# Autodesk Inventor assembly: FulBotV2P1
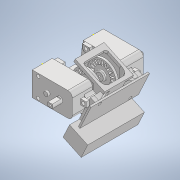
[picture p0: Inventor's stored thumbnail of the model, 180x180]
Saved by Autodesk Inventor 2022 (Build 260153070, 153G)
## iProperties
Created: 2022-02-15
Part Number: FulBotV2P1
Document SubType Name: Assembly
Designer: a laptop
Author: a laptop
## Documents named in this file (6)
- C:\Users\a laptop\Desktop\SumoBot\FulBotV2P1.iam
- C:\Users\a laptop\Desktop\SumoBot\sumobotENCODER\EncoderV2\EncoderV2.5.iam
- C:\Users\a laptop\Desktop\SumoBot\REF_PART\2sLIPO_SMALLER.ipt
- C:\Users\a laptop\Desktop\SumoBot\sumobotENCODER\EncoderV2\EncoderV2.5_MIR.iam
- C:\Users\a laptop\Desktop\SumoBot\REF_PART\XL4015.ipt
- C:\Users\a laptop\Desktop\SumoBot\sumobotFRAME\Encoderconnector.ipt
## Components (5 placed, 5 different names)
1. EncoderV2.5:1 [sub-assembly] — Flush:2, Flush:3, Mate:1, Mate:4
2. 2sLIPO_SMALLER:1 — Mate:3
3. EncoderV2.5_MIR:1 [sub-assembly] — Flush:2, Flush:3, Mate:2
4. XL4015:1 — Mate:5, Mate:6, Mate:7
5. Encoderconnector:1 — Mate:1, Mate:2, Mate:3, Mate:4, Mate:5, Mate:6, Mate:7
## Relationships (9: Mate 7, Flush 2)
- Flush:2: EncoderV2.5:1 ↔ EncoderV2.5_MIR:1
- Flush:3: EncoderV2.5:1 ↔ EncoderV2.5_MIR:1
- Mate:1: EncoderV2.5:1 ↔ Encoderconnector:1
- Mate:2: EncoderV2.5_MIR:1 ↔ Encoderconnector:1
- Mate:3: 2sLIPO_SMALLER:1 ↔ Encoderconnector:1
- Mate:4: EncoderV2.5:1 ↔ Encoderconnector:1
- Mate:5: XL4015:1 ↔ Encoderconnector:1
- Mate:6: XL4015:1 ↔ Encoderconnector:1
- Mate:7: XL4015:1 ↔ Encoderconnector:1
